# Autodesk Inventor assembly: Carriage Streamlined
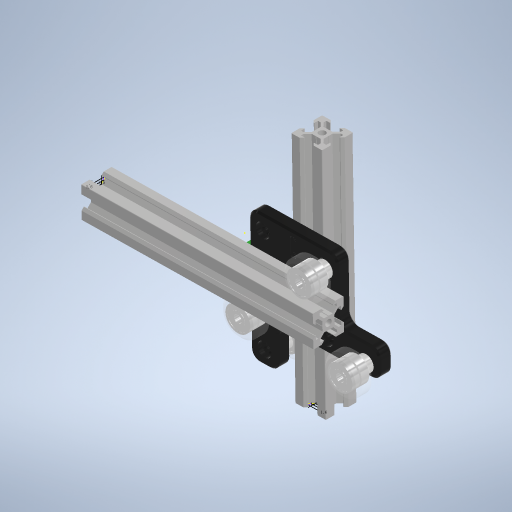
[picture p0: Inventor's stored thumbnail of the model, 512x512]
Saved by Autodesk Inventor 2024 (Build 280153000, 153)
## iProperties
Created: 2022-12-12
Part Number: Carriage Streamlined
Document SubType Name: Assembly
Designer: AdminForWorker
Title: Carriage Streamlined v19
Author: AdminForWorker
## Documents named in this file (13)
- C:\Users\lunima\Desktop\DOSYN\IPT\Carriage\Carriage Streamlined.iam
- C:\Users\lunima\Desktop\DOSYN\IPT\Carriage\Routed Spacer.ipt
- C:\Users\lunima\Desktop\DOSYN\IPT\Carriage\Wheel.iam
- C:\Users\lunima\Desktop\DOSYN\IPT\Carriage\Wheel_1.iam
- C:\Users\lunima\Desktop\DOSYN\IPT\Carriage\Wheel_2.iam
- C:\Users\lunima\Desktop\DOSYN\IPT\Carriage\Wheel_3.iam
- C:\Users\lunima\Desktop\DOSYN\IPT\Carriage\Wheel_4.iam
- C:\Users\lunima\Desktop\DOSYN\IPT\Carriage\Wheel_5.iam
- C:\Users\lunima\Desktop\DOSYN\IPT\Carriage\Carriage.ipt
- C:\Users\lunima\Desktop\DOSYN\IPT\Carriage\Component8.ipt
- C:\Users\lunima\Desktop\DOSYN\IPT\Carriage\Belt Clip.ipt
- C:\Users\lunima\Desktop\DOSYN\IPT\Carriage\Pogo Pin Clip.ipt
- C:\Users\lunima\Desktop\DOSYN\IPT\Main Structure\2020.ipt
## Components (18 placed, 7 different names)
1. Routed Spacer:1
2. Routed Spacer:2
3. Wheel:1 [sub-assembly]
4. Wheel:2 [sub-assembly]
5. Wheel:3 [sub-assembly]
6. Routed Spacer:4
7. Routed Spacer:5
8. Routed Spacer:6
9. Wheel:4 [sub-assembly]
10. Wheel:5 [sub-assembly]
11. Wheel:6 [sub-assembly]
12. Carriage:1 — 旋转:1, 旋转:2, 配合:1, 表面齐平:1, 旋转:3, 配合:2, 表面齐平:2
13. Component8:1
14. Belt Clip:1 — 旋转:1
15. Pogo Pin Clip:1 — 旋转:2
16. Pogo Pin Clip:2 — 旋转:3
17. 2020:1 — 配合:1, 表面齐平:1
18. 2020:2 — 配合:2, 表面齐平:2
## Relationships (7: RevoluteJoint 3, Mate 2, Flush 2)
- 旋转:1 [RevoluteJoint]: Carriage:1 ↔ Belt Clip:1
- 旋转:2 [RevoluteJoint]: Carriage:1 ↔ Pogo Pin Clip:1
- 配合:1 [Mate] (1.5 mm): Carriage:1 ↔ 2020:1
- 表面齐平:1 [Flush] (18.85 mm): Carriage:1 ↔ 2020:1
- 旋转:3 [RevoluteJoint]: Carriage:1 ↔ Pogo Pin Clip:2
- 配合:2 [Mate] (1.5 mm): Carriage:1 ↔ 2020:2
- 表面齐平:2 [Flush] (18.85 mm): Carriage:1 ↔ 2020:2
